# Autodesk Inventor assembly: TestAssm
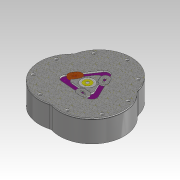
[picture p0: Inventor's stored thumbnail of the model, 180x180]
Saved by Autodesk Inventor 2020 (Build 240168000, 168)
## iProperties
Created: 2021-05-17
Part Number: TestAssm
Document SubType Name: Assembly
Designer: DDeGo
Author: DDeGo
## Documents named in this file (14)
- C:\Users\DDeGo\Documents\Drew\Projects\AirWankelEngine\cad\LiquidPiston V1\TestAssm.iam
- C:\Users\DDeGo\Documents\Drew\Projects\AirWankelEngine\cad\LiquidPiston V1\TestHousing.ipt
- C:\Users\DDeGo\Documents\Drew\Projects\AirWankelEngine\cad\LiquidPiston V1\TestRotor.ipt
- C:\Users\DDeGo\Documents\Drew\Projects\AirWankelEngine\cad\LiquidPiston V1\TestCam.ipt
- C:\Users\DDeGo\Documents\Drew\Projects\AirWankelEngine\cad\LiquidPiston V1\TestAssm\Design Accelerator\Spur Gears1.iam
- C:\Users\DDeGo\Documents\Drew\Projects\AirWankelEngine\cad\hardware\6701 bearing.ipt
- C:\Users\DDeGo\Documents\Drew\Projects\AirWankelEngine\cad\LiquidPiston V1\TestHead.ipt
- C:\Users\DDeGo\Documents\Drew\Projects\AirWankelEngine\cad\LiquidPiston V1\ApexSeal.ipt
- C:\Users\DDeGo\Documents\Drew\Projects\AirWankelEngine\cad\hardware\MR85 bearing.ipt
- C:\Users\DDeGo\Documents\Drew\Projects\AirWankelEngine\cad\LiquidPiston V1\TestRotorTeeth.ipt
- C:\Users\DDeGo\Documents\Drew\Projects\AirWankelEngine\cad\LiquidPiston V1\Flywheel.ipt
- C:\Users\DDeGo\Documents\Drew\Projects\AirWankelEngine\cad\hardware\oring_4x2x1.ipt
- C:\Users\DDeGo\Documents\Drew\Projects\AirWankelEngine\cad\LiquidPiston V1\ValveThing.ipt
- C:\Users\DDeGo\Documents\Drew\Projects\AirWankelEngine\cad\hardware\2x22 pin.ipt
## Components (20 placed, 13 different names)
1. TestHousing:1 — Mate:2, Mate:11, Mate:14, Mate:15, Mate:20, Mate:21, Mate:65, Mate:66, Mate:67, Mate:68, Mate:69
2. TestRotor:1 — Mate:2, Mate:3, Rotation:1, Mate:5, Mate:29, Mate:30, Angle:1, Mate:42, Mate:57
3. TestCam:1 — Mate:3, Rotation:1, Mate:43, Mate:44, Mate:46, Mate:47, Mate:48, Flush:6
4. Spur Gears:1 [sub-assembly]
5. 6701 bearing:1 — Mate:5, Mate:42, Flush:6
6. ApexSeal:1 — Mate:11, Mate:67
7. ApexSeal:2 — Mate:14, Mate:68
8. ApexSeal:3 — Mate:15, Mate:66
9. MR85 bearing:1 — Mate:20, Mate:21, Mate:32, Mate:33
10. MR85 bearing:2 — Mate:46, Mate:48, Mate:64
11. TestRotorTeeth:1 — Mate:29, Mate:30, Angle:1
12. Flywheel:1 — Mate:32, Mate:33, Mate:45, Mate:47
13. oring_4x2x1:1 — Flush:2, Flush:3, Mate:56, Mate:63, Tangent:1
14. oring_4x2x1:2 — Flush:2, Mate:55, Mate:61
15. oring_4x2x1:3 — Flush:3, Mate:62
16. ValveThing:1 — Flush:4, Flush:5, Mate:57, Mate:58, Angle:3, Mate:63, Tangent:1
17. ValveThing:2 — Flush:4, Mate:56, Mate:59, Angle:4, Mate:62
18. ValveThing:3 — Flush:5, Mate:55, Mate:60, Angle:2, Mate:61
19. 2x22 pin:1 — Mate:43, Mate:44, Mate:45
20. TestHead:1 — Mate:58, Mate:59, Mate:60, Angle:2, Angle:3, Angle:4, Mate:64, Mate:65, Mate:69
## Relationships (45: Mate 34, Flush 5, Angle 4, RelateRotation 1, Tangent 1)
- Mate:2 (-0.25 mm): TestHousing:1 ↔ TestRotor:1
- Mate:3: TestRotor:1 ↔ TestCam:1
- Rotation:1 [RelateRotation] (2 ul): TestRotor:1 ↔ TestCam:1
- Mate:5: TestRotor:1 ↔ 6701 bearing:1
- Mate:11 (0.1 mm): TestHousing:1 ↔ ApexSeal:1
- Mate:14 (0.1 mm): TestHousing:1 ↔ ApexSeal:2
- Mate:15 (0.1 mm): TestHousing:1 ↔ ApexSeal:3
- Mate:20: TestHousing:1 ↔ MR85 bearing:1
- Mate:21: TestHousing:1 ↔ MR85 bearing:1
- Mate:29: TestRotor:1 ↔ TestRotorTeeth:1
- Mate:30: TestRotor:1 ↔ TestRotorTeeth:1
- Angle:1 (0 deg): TestRotor:1 ↔ TestRotorTeeth:1
- Mate:32: MR85 bearing:1 ↔ Flywheel:1
- Mate:33: MR85 bearing:1 ↔ Flywheel:1
- Flush:2: oring_4x2x1:1 ↔ oring_4x2x1:2
- Flush:3: oring_4x2x1:1 ↔ oring_4x2x1:3
- Flush:4: ValveThing:1 ↔ ValveThing:2
- Flush:5: ValveThing:1 ↔ ValveThing:3
- Mate:42: TestRotor:1 ↔ 6701 bearing:1
- Mate:43: TestCam:1 ↔ 2x22 pin:1
- Mate:44: TestCam:1 ↔ 2x22 pin:1
- Mate:45: Flywheel:1 ↔ 2x22 pin:1
- Mate:46: TestCam:1 ↔ MR85 bearing:2
- Mate:47: TestCam:1 ↔ Flywheel:1
- Mate:48: TestCam:1 ↔ MR85 bearing:2
- Mate:55: oring_4x2x1:2 ↔ ValveThing:3
- Mate:56: oring_4x2x1:1 ↔ ValveThing:2
- Flush:6: TestCam:1 ↔ 6701 bearing:1
- Mate:57: TestRotor:1 ↔ ValveThing:1
- Mate:58: ValveThing:1 ↔ TestHead:1
- Mate:59: ValveThing:2 ↔ TestHead:1
- Mate:60: ValveThing:3 ↔ TestHead:1
- Angle:2 (0 deg): ValveThing:3 ↔ TestHead:1
- Angle:3 (0 deg): ValveThing:1 ↔ TestHead:1
- Angle:4 (0 deg): ValveThing:2 ↔ TestHead:1
- Mate:61: oring_4x2x1:2 ↔ ValveThing:3
- Mate:62: oring_4x2x1:3 ↔ ValveThing:2
- Mate:63: oring_4x2x1:1 ↔ ValveThing:1
- Tangent:1: oring_4x2x1:1 ↔ ValveThing:1
- Mate:64: MR85 bearing:2 ↔ TestHead:1
- Mate:65: TestHousing:1 ↔ TestHead:1
- Mate:66: TestHousing:1 ↔ ApexSeal:3
- Mate:67: TestHousing:1 ↔ ApexSeal:1
- Mate:68: TestHousing:1 ↔ ApexSeal:2
- Mate:69: TestHousing:1 ↔ TestHead:1
